# Autodesk Inventor assembly: CAM1
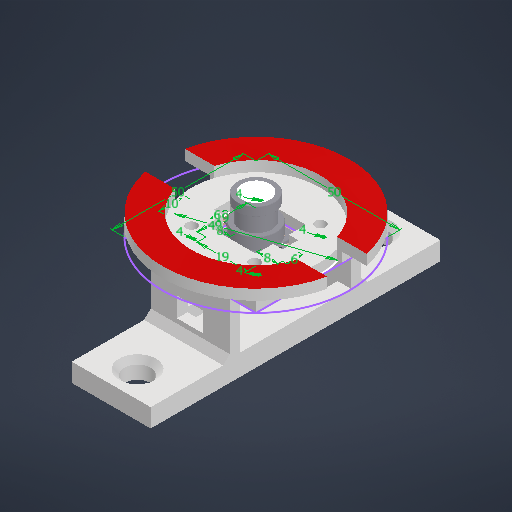
[picture p0: Inventor's stored thumbnail of the model, 512x512]
Saved by Autodesk Inventor 2026.2 (Build 302298000, 298)
## iProperties
Created: 2025-12-02
Part Number: CAM1
Document SubType Name: Assembly
Designer: alexa
Author: alexa
## Documents named in this file (3)
- C:\Users\alexa\Desktop\DA\CAM1.iam
- F:\07_Diplomarbeit\FIT0892\FIT0892\FIT0892.iam
- C:\Users\alexa\Desktop\CAM1.ipt
## Components (2 placed, 2 different names)
1. FIT0892:1 [sub-assembly] — Fluchtend:5
2. CAM1:1 — Fluchtend:4, Fluchtend:5
## Relationships (3: Flush 3)
- Fluchtend:3 [Flush] (-5 mm)
- Fluchtend:4 [Flush]: CAM1:1
- Fluchtend:5 [Flush]: FIT0892:1 ↔ CAM1:1
## Named parameters: Finish1_Area = 17.1195
note: some values were not read from the file. Shown as the stored number, unit unknown: "Finish1_Area".
